# Autodesk Inventor assembly: RobotGripper
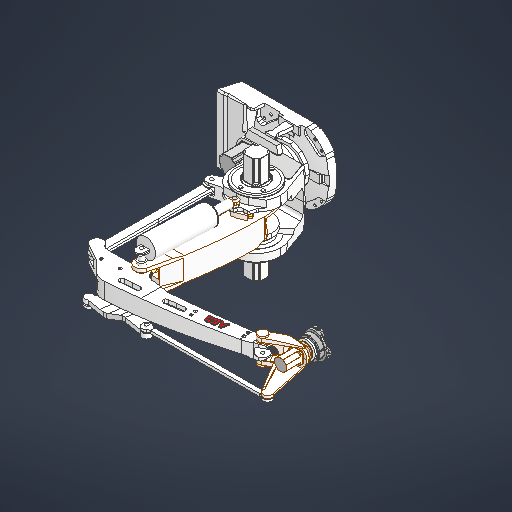
[picture p0: Inventor's stored thumbnail of the model, 512x512]
Saved by Autodesk Inventor 2026.2 (Build 302298000, 298)
## iProperties
Created: 2025-11-24
Part Number: RobotGripper
Document SubType Name: Assembly
Designer: USUARIO
Author: USUARIO
## Documents named in this file (3)
- F:\UNAL\14. SEMESTRE\AUTOMATIZACIÓN DE PROCESOS DE MANUFACTURA\GitHub\Los4Automaticos\CAD\InventorProyecto\RobotGripper.iam
- F:\UNAL\14. SEMESTRE\AUTOMATIZACIÓN DE PROCESOS DE MANUFACTURA\GitHub\Los4Automaticos\CAD\InventorProyecto\Robot.ipt
- F:\UNAL\14. SEMESTRE\AUTOMATIZACIÓN DE PROCESOS DE MANUFACTURA\GitHub\Los4Automaticos\CAD\InventorProyecto\GripperOnePiece.ipt
## Components (2 placed, 2 different names)
1. Robot:1 — Cilíndrica:1, Coincidencia:1
2. GripperOnePiece:1 — Cilíndrica:1, Coincidencia:1
## Relationships (2: CylindricalJoint 1, Mate 1)
- Cilíndrica:1 [CylindricalJoint]: Robot:1 ↔ GripperOnePiece:1
- Coincidencia:1 [Mate]: Robot:1 ↔ GripperOnePiece:1
